# Autodesk Inventor assembly: F-wing
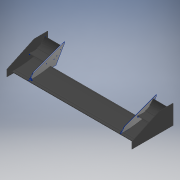
[picture p0: Inventor's stored thumbnail of the model, 180x180]
Saved by Autodesk Inventor 2018.1 (Build 221171000, 171)
## iProperties
Created: 2017-10-22
Part Number: F-wing
Material: 一般
Document SubType Name: Assembly
Designer: ku_sk
Mass: 4009.03 g
Surface Area: 15231.2 cm^2
Volume: 2840.08 cm^3
Density: 1.41159 g/cm^3
Author: ku_sk
## Documents named in this file (6)
- D:\kuwano\Documents\Inventor\KITformula\KS-15_Aero_CAD\type4\F-wing\F-wing.iam
- D:\kuwano\Documents\Inventor\KITformula\KS-15_Aero_CAD\type4\F-wing\parts\element_side\element_L.iam
- D:\kuwano\Documents\Inventor\KITformula\KS-15_Aero_CAD\type4\F-wing\parts\element_side\element_R.iam
- D:\kuwano\Documents\Inventor\KITformula\KS-15_Aero_CAD\type4\F-wing\parts\base\base_booled.ipt
- D:\kuwano\Documents\Inventor\KITformula\KS-15_Aero_CAD\type4\F-wing\parts\side.ipt
- D:\kuwano\Documents\Inventor\KITformula\KS-15_Aero_CAD\type4\F-wing\parts\element_clip.ipt
## Components (17 placed, 5 different names)
1. element_L:1 [sub-assembly] — メイト:5, メイト:6, メイト:7, メイト:41, メイト:49
2. element_R:1 [sub-assembly] — メイト:2, メイト:3, メイト:4, メイト:38, メイト:52
3. base_booled:1 — メイト:2, メイト:3, メイト:4, メイト:5, メイト:6, メイト:7, メイト:12, メイト:13, フラッシュ:3, フラッシュ:4, フラッシュ:5, フラッシュ:6, メイト:14, メイト:15, メイト:16, メイト:17, メイト:22, メイト:23, メイト:24, メイト:25, メイト:26, メイト:27, メイト:30, メイト:31, メイト:34, メイト:35, メイト:36, メイト:37, メイト:43, メイト:45, メイト:46, メイト:47, メイト:48, メイト:50, メイト:51, メイト:53
4. side:1 — メイト:12, フラッシュ:3, フラッシュ:5, メイト:18, メイト:19, メイト:28, メイト:29
5. side:2 — メイト:13, フラッシュ:4, フラッシュ:6, メイト:20, メイト:21, メイト:32, メイト:33
6. element_clip:1 — メイト:16, メイト:19, メイト:23
7. element_clip:2 — メイト:17, メイト:18, メイト:24
8. element_clip:3 — メイト:14, メイト:20, メイト:25
9. element_clip:4 — メイト:15, メイト:21, メイト:22
10. element_clip:5 — メイト:30, メイト:33, メイト:35
11. element_clip:6 — メイト:31, メイト:32, メイト:34
12. element_clip:7 — メイト:26, メイト:29, メイト:36
13. element_clip:8 — メイト:27, メイト:28, メイト:37
14. element_clip:11 — メイト:38, メイト:45, メイト:46
15. element_clip:12 — メイト:41, メイト:43, メイト:47
16. element_clip:13 — メイト:48, メイト:49, メイト:50
17. element_clip:14 — メイト:51, メイト:52, メイト:53
## Relationships (48: Mate 44, Flush 4)
- メイト:2 [Mate]: element_R:1 ↔ base_booled:1
- メイト:3 [Mate]: element_R:1 ↔ base_booled:1
- メイト:4 [Mate]: element_R:1 ↔ base_booled:1
- メイト:5 [Mate]: element_L:1 ↔ base_booled:1
- メイト:6 [Mate]: element_L:1 ↔ base_booled:1
- メイト:7 [Mate]: element_L:1 ↔ base_booled:1
- メイト:12 [Mate]: base_booled:1 ↔ side:1
- メイト:13 [Mate]: base_booled:1 ↔ side:2
- フラッシュ:3 [Flush] (-20 mm): base_booled:1 ↔ side:1
- フラッシュ:4 [Flush] (20 mm): base_booled:1 ↔ side:2
- フラッシュ:5 [Flush] (55 mm): base_booled:1 ↔ side:1
- フラッシュ:6 [Flush] (55 mm): base_booled:1 ↔ side:2
- メイト:14 [Mate]: base_booled:1 ↔ element_clip:3
- メイト:15 [Mate]: base_booled:1 ↔ element_clip:4
- メイト:16 [Mate]: base_booled:1 ↔ element_clip:1
- メイト:17 [Mate]: base_booled:1 ↔ element_clip:2
- メイト:18 [Mate]: side:1 ↔ element_clip:2
- メイト:19 [Mate]: side:1 ↔ element_clip:1
- メイト:20 [Mate]: side:2 ↔ element_clip:3
- メイト:21 [Mate]: side:2 ↔ element_clip:4
- メイト:22 [Mate]: base_booled:1 ↔ element_clip:4
- メイト:23 [Mate]: base_booled:1 ↔ element_clip:1
- メイト:24 [Mate]: base_booled:1 ↔ element_clip:2
- メイト:25 [Mate]: base_booled:1 ↔ element_clip:3
- メイト:26 [Mate]: base_booled:1 ↔ element_clip:7
- メイト:27 [Mate]: base_booled:1 ↔ element_clip:8
- メイト:28 [Mate]: side:1 ↔ element_clip:8
- メイト:29 [Mate]: side:1 ↔ element_clip:7
- メイト:30 [Mate]: base_booled:1 ↔ element_clip:5
- メイト:31 [Mate]: base_booled:1 ↔ element_clip:6
- メイト:32 [Mate]: side:2 ↔ element_clip:6
- メイト:33 [Mate]: side:2 ↔ element_clip:5
- メイト:34 [Mate]: base_booled:1 ↔ element_clip:6
- メイト:35 [Mate]: base_booled:1 ↔ element_clip:5
- メイト:36 [Mate]: base_booled:1 ↔ element_clip:7
- メイト:37 [Mate]: base_booled:1 ↔ element_clip:8
- メイト:38 [Mate]: element_R:1 ↔ element_clip:11
- メイト:41 [Mate]: element_L:1 ↔ element_clip:12
- メイト:43 [Mate]: base_booled:1 ↔ element_clip:12
- メイト:45 [Mate]: base_booled:1 ↔ element_clip:11
- メイト:46 [Mate]: base_booled:1 ↔ element_clip:11
- メイト:47 [Mate]: base_booled:1 ↔ element_clip:12
- メイト:48 [Mate]: base_booled:1 ↔ element_clip:13
- メイト:49 [Mate]: element_L:1 ↔ element_clip:13
- メイト:50 [Mate]: base_booled:1 ↔ element_clip:13
- メイト:51 [Mate]: base_booled:1 ↔ element_clip:14
- メイト:52 [Mate]: element_R:1 ↔ element_clip:14
- メイト:53 [Mate]: base_booled:1 ↔ element_clip:14
